# Autodesk Inventor assembly: FinalRobot-ver4-1111-2021
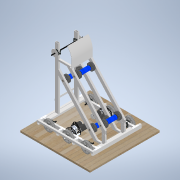
[picture p0: Inventor's stored thumbnail of the model, 180x180]
Saved by Autodesk Inventor 2020 (Build 240168000, 168)
## iProperties
Created: 2021-01-26
Part Number: FinalRobot-ver4-1111-2021
Document SubType Name: Assembly
Designer: Caitlin
Author: Caitlin
## Documents named in this file (7)
- D:\PHRC CADD 2021\PHRC CADD\2020 Infinite Recharge\2021 Infinite Recharge\FinalRobot-ver4-1111-2021.iam
- D:\PHRC CADD 2021\PHRC CADD\2020 Infinite Recharge\2021 Infinite Recharge\Chassis\Chassis-ver1-1111-2021.iam
- D:\PHRC CADD 2021\PHRC CADD\2020 Infinite Recharge\Platform.ver1-1111-2020.ipt
- D:\PHRC CADD 2021\PHRC CADD\2020 Infinite Recharge\Storage\Assemblies\StorageAssembly.ver4-1111-2020.iam
- D:\PHRC CADD 2021\PHRC CADD\2020 Infinite Recharge\Shooting\Assemblies\ShooterPrototype-ver2-1111-2019.iam
- D:\PHRC CADD 2021\PHRC CADD\Resources\VEXpro Resources\Bearings\0.5inHexFlangedBearing(1.125inx0.313in)-1111-2016.ipt
- D:\PHRC CADD 2021\PHRC CADD\2020 Infinite Recharge\2021 Infinite Recharge\Chassis\Roller-ver4-1111-2021.iam
## Components (24 placed, 6 different names)
1. Chassis-ver1-1111-2021:1 [sub-assembly] — Mate:1, Angle:1, Flush:1, Flush:2, Mate:2, Mate:3, Mate:4, Mate:5, Mate:6, Flush:3
2. Platform.ver1-1111-2020:1 — Mate:1, Angle:1, Flush:1, Flush:2
3. StorageAssembly.ver4-1111-2020:1 [sub-assembly] — Mate:2, Mate:3, Mate:4, Cylindrical:1, Mate:7, Cylindrical:2, Mate:8, Cylindrical:3, Mate:9, Cylindrical:4, Mate:10, Cylindrical:5, Mate:11, Cylindrical:6, Mate:12, Cylindrical:7, Mate:13, Cylindrical:8, Mate:14, Cylindrical:9, Mate:15, Cylindrical:10, Mate:16, Cylindrical:11, Mate:17, Cylindrical:12, Mate:18, Cylindrical:13, Mate:19, Cylindrical:14, Mate:20, Cylindrical:15, Mate:21, Cylindrical:16, Mate:22, Flush:4, Flush:5, Flush:6, Flush:7
4. ShooterPrototype-ver2-1111-2019:1 [sub-assembly] — Mate:5, Mate:6, Flush:3
5. 0.5inHexFlangedBearing(1.125inx0.313in)-1111-2016:1 — Cylindrical:1, Mate:7, Cylindrical:20
6. 0.5inHexFlangedBearing(1.125inx0.313in)-1111-2016:2 — Cylindrical:2, Mate:8, Cylindrical:19
7. 0.5inHexFlangedBearing(1.125inx0.313in)-1111-2016:3 — Cylindrical:3, Mate:9, Cylindrical:17
8. 0.5inHexFlangedBearing(1.125inx0.313in)-1111-2016:4 — Cylindrical:4, Mate:10, Cylindrical:18
9. 0.5inHexFlangedBearing(1.125inx0.313in)-1111-2016:5 — Cylindrical:5, Mate:11
10. 0.5inHexFlangedBearing(1.125inx0.313in)-1111-2016:6 — Cylindrical:6, Mate:12
11. 0.5inHexFlangedBearing(1.125inx0.313in)-1111-2016:7 — Cylindrical:7, Mate:13
12. 0.5inHexFlangedBearing(1.125inx0.313in)-1111-2016:8 — Cylindrical:8, Mate:14
13. 0.5inHexFlangedBearing(1.125inx0.313in)-1111-2016:9 — Cylindrical:9, Mate:15
14. 0.5inHexFlangedBearing(1.125inx0.313in)-1111-2016:10 — Cylindrical:10, Mate:16
15. 0.5inHexFlangedBearing(1.125inx0.313in)-1111-2016:11 — Cylindrical:11, Mate:17
16. 0.5inHexFlangedBearing(1.125inx0.313in)-1111-2016:12 — Cylindrical:12, Mate:18
17. 0.5inHexFlangedBearing(1.125inx0.313in)-1111-2016:13 — Cylindrical:13, Mate:19
18. 0.5inHexFlangedBearing(1.125inx0.313in)-1111-2016:14 — Cylindrical:14, Mate:20
19. 0.5inHexFlangedBearing(1.125inx0.313in)-1111-2016:15 — Cylindrical:15, Mate:21
20. 0.5inHexFlangedBearing(1.125inx0.313in)-1111-2016:16 — Cylindrical:16, Mate:22
21. Roller-ver4-1111-2021:1 [sub-assembly] — Cylindrical:17, Flush:4
22. Roller-ver4-1111-2021:2 [sub-assembly] — Cylindrical:18, Flush:5
23. Roller-ver4-1111-2021:3 [sub-assembly] — Cylindrical:19, Flush:6
24. Roller-ver4-1111-2021:4 [sub-assembly] — Cylindrical:20, Flush:7
## Relationships (50: Mate 22, CylindricalJoint 20, Flush 7, Angle 1)
- Mate:1 (47.625 mm): Chassis-ver1-1111-2021:1 ↔ Platform.ver1-1111-2020:1
- Angle:1 (0 deg): Chassis-ver1-1111-2021:1 ↔ Platform.ver1-1111-2020:1
- Flush:1 (152.4 mm): Chassis-ver1-1111-2021:1 ↔ Platform.ver1-1111-2020:1
- Flush:2 (114.3 mm): Chassis-ver1-1111-2021:1 ↔ Platform.ver1-1111-2020:1
- Mate:2: Chassis-ver1-1111-2021:1 ↔ StorageAssembly.ver4-1111-2020:1
- Mate:3: Chassis-ver1-1111-2021:1 ↔ StorageAssembly.ver4-1111-2020:1
- Mate:4: Chassis-ver1-1111-2021:1 ↔ StorageAssembly.ver4-1111-2020:1
- Mate:5: Chassis-ver1-1111-2021:1 ↔ ShooterPrototype-ver2-1111-2019:1
- Mate:6: Chassis-ver1-1111-2021:1 ↔ ShooterPrototype-ver2-1111-2019:1
- Flush:3: Chassis-ver1-1111-2021:1 ↔ ShooterPrototype-ver2-1111-2019:1
- Cylindrical:1: StorageAssembly.ver4-1111-2020:1 ↔ 0.5inHexFlangedBearing(1.125inx0.313in)-1111-2016:1
- Mate:7: StorageAssembly.ver4-1111-2020:1 ↔ 0.5inHexFlangedBearing(1.125inx0.313in)-1111-2016:1
- Cylindrical:2: StorageAssembly.ver4-1111-2020:1 ↔ 0.5inHexFlangedBearing(1.125inx0.313in)-1111-2016:2
- Mate:8: StorageAssembly.ver4-1111-2020:1 ↔ 0.5inHexFlangedBearing(1.125inx0.313in)-1111-2016:2
- Cylindrical:3: StorageAssembly.ver4-1111-2020:1 ↔ 0.5inHexFlangedBearing(1.125inx0.313in)-1111-2016:3
- Mate:9: StorageAssembly.ver4-1111-2020:1 ↔ 0.5inHexFlangedBearing(1.125inx0.313in)-1111-2016:3
- Cylindrical:4: StorageAssembly.ver4-1111-2020:1 ↔ 0.5inHexFlangedBearing(1.125inx0.313in)-1111-2016:4
- Mate:10: StorageAssembly.ver4-1111-2020:1 ↔ 0.5inHexFlangedBearing(1.125inx0.313in)-1111-2016:4
- Cylindrical:5: StorageAssembly.ver4-1111-2020:1 ↔ 0.5inHexFlangedBearing(1.125inx0.313in)-1111-2016:5
- Mate:11: StorageAssembly.ver4-1111-2020:1 ↔ 0.5inHexFlangedBearing(1.125inx0.313in)-1111-2016:5
- Cylindrical:6: StorageAssembly.ver4-1111-2020:1 ↔ 0.5inHexFlangedBearing(1.125inx0.313in)-1111-2016:6
- Mate:12: StorageAssembly.ver4-1111-2020:1 ↔ 0.5inHexFlangedBearing(1.125inx0.313in)-1111-2016:6
- Cylindrical:7: StorageAssembly.ver4-1111-2020:1 ↔ 0.5inHexFlangedBearing(1.125inx0.313in)-1111-2016:7
- Mate:13: StorageAssembly.ver4-1111-2020:1 ↔ 0.5inHexFlangedBearing(1.125inx0.313in)-1111-2016:7
- Cylindrical:8: StorageAssembly.ver4-1111-2020:1 ↔ 0.5inHexFlangedBearing(1.125inx0.313in)-1111-2016:8
- Mate:14: StorageAssembly.ver4-1111-2020:1 ↔ 0.5inHexFlangedBearing(1.125inx0.313in)-1111-2016:8
- Cylindrical:9: StorageAssembly.ver4-1111-2020:1 ↔ 0.5inHexFlangedBearing(1.125inx0.313in)-1111-2016:9
- Mate:15: StorageAssembly.ver4-1111-2020:1 ↔ 0.5inHexFlangedBearing(1.125inx0.313in)-1111-2016:9
- Cylindrical:10: StorageAssembly.ver4-1111-2020:1 ↔ 0.5inHexFlangedBearing(1.125inx0.313in)-1111-2016:10
- Mate:16: StorageAssembly.ver4-1111-2020:1 ↔ 0.5inHexFlangedBearing(1.125inx0.313in)-1111-2016:10
- Cylindrical:11: StorageAssembly.ver4-1111-2020:1 ↔ 0.5inHexFlangedBearing(1.125inx0.313in)-1111-2016:11
- Mate:17: StorageAssembly.ver4-1111-2020:1 ↔ 0.5inHexFlangedBearing(1.125inx0.313in)-1111-2016:11
- Cylindrical:12: StorageAssembly.ver4-1111-2020:1 ↔ 0.5inHexFlangedBearing(1.125inx0.313in)-1111-2016:12
- Mate:18: StorageAssembly.ver4-1111-2020:1 ↔ 0.5inHexFlangedBearing(1.125inx0.313in)-1111-2016:12
- Cylindrical:13: StorageAssembly.ver4-1111-2020:1 ↔ 0.5inHexFlangedBearing(1.125inx0.313in)-1111-2016:13
- Mate:19: StorageAssembly.ver4-1111-2020:1 ↔ 0.5inHexFlangedBearing(1.125inx0.313in)-1111-2016:13
- Cylindrical:14: StorageAssembly.ver4-1111-2020:1 ↔ 0.5inHexFlangedBearing(1.125inx0.313in)-1111-2016:14
- Mate:20: StorageAssembly.ver4-1111-2020:1 ↔ 0.5inHexFlangedBearing(1.125inx0.313in)-1111-2016:14
- Cylindrical:15: StorageAssembly.ver4-1111-2020:1 ↔ 0.5inHexFlangedBearing(1.125inx0.313in)-1111-2016:15
- Mate:21: StorageAssembly.ver4-1111-2020:1 ↔ 0.5inHexFlangedBearing(1.125inx0.313in)-1111-2016:15
- Cylindrical:16: StorageAssembly.ver4-1111-2020:1 ↔ 0.5inHexFlangedBearing(1.125inx0.313in)-1111-2016:16
- Mate:22: StorageAssembly.ver4-1111-2020:1 ↔ 0.5inHexFlangedBearing(1.125inx0.313in)-1111-2016:16
- Cylindrical:17: 0.5inHexFlangedBearing(1.125inx0.313in)-1111-2016:3 ↔ Roller-ver4-1111-2021:1
- Flush:4: StorageAssembly.ver4-1111-2020:1 ↔ Roller-ver4-1111-2021:1
- Cylindrical:18: 0.5inHexFlangedBearing(1.125inx0.313in)-1111-2016:4 ↔ Roller-ver4-1111-2021:2
- Flush:5: StorageAssembly.ver4-1111-2020:1 ↔ Roller-ver4-1111-2021:2
- Cylindrical:19: 0.5inHexFlangedBearing(1.125inx0.313in)-1111-2016:2 ↔ Roller-ver4-1111-2021:3
- Flush:6: StorageAssembly.ver4-1111-2020:1 ↔ Roller-ver4-1111-2021:3
- Cylindrical:20: 0.5inHexFlangedBearing(1.125inx0.313in)-1111-2016:1 ↔ Roller-ver4-1111-2021:4
- Flush:7: StorageAssembly.ver4-1111-2020:1 ↔ Roller-ver4-1111-2021:4
